# Autodesk Inventor assembly: new_U64_shoulder_with_offset
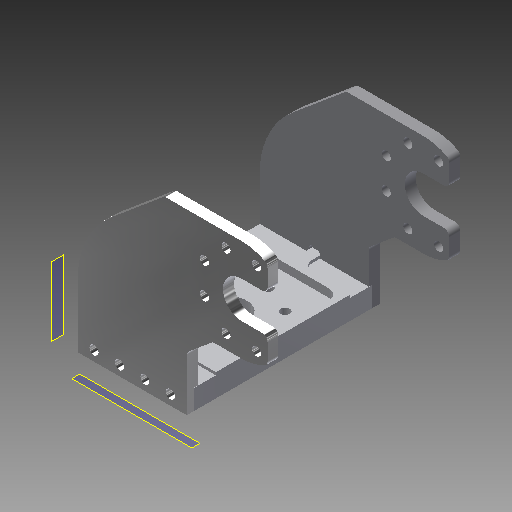
[picture p0: Inventor's stored thumbnail of the model, 512x512]
Saved by Autodesk Inventor 2018 (Build 220112000, 112)
## iProperties
Created: 2018-04-10
Part Number: new_U64_shoulder_with_offset
Document SubType Name: Assembly
Designer: medrimonia
Author: medrimonia
## Documents named in this file (4)
- C:\Users\etd\Dropbox\SigmaBan\SigmaBanV2.1\new_U\new_U64_shoulder_with_offset.iam
- C:\Users\etd\Dropbox\SigmaBan\SigmaBanV2.1\new_U\new_side_u64_shoulder.ipt
- C:\Users\etd\Dropbox\SigmaBan\SigmaBanV2.1\new_base_u64_long.ipt
- C:\Users\etd\Dropbox\SigmaBan\SigmaBanV2.1\new_U\new_side_u64_shoulder_MIR.ipt
## Components (3 placed, 3 different names)
1. new_side_u64_shoulder:1 — Mate:2, Mate:3
2. new_base_u64_long:1 — Mate:2, Mate:3
3. new_side_u64_shoulder_MIR:1
## Relationships (2: Mate 2)
- Mate:2: new_side_u64_shoulder:1 ↔ new_base_u64_long:1
- Mate:3: new_side_u64_shoulder:1 ↔ new_base_u64_long:1
